# Autodesk Inventor assembly: link1
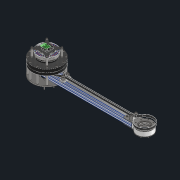
[picture p0: Inventor's stored thumbnail of the model, 180x180]
Saved by Autodesk Inventor 2022 (Build 260153000, 153)
## iProperties
Created: 2021-10-13
Part Number: link1
Document SubType Name: Assembly
Designer: Yuta Kage
Author: Yuta Kage
## Documents named in this file (2)
- C:\Users\yuta0\Documents\GitHub\catchrobo_hardware\mesh\scara\link1.iam
- C:\Users\yuta0\Documents\GitHub\catchrobo_hardware\assy-scara\s-assy-scara_link1.iam
## Components (1 placed, 1 different names)
1. s-assy-scara_link1:1 [sub-assembly] — メイト:1, メイト:2, メイト:3
## Relationships (3: Mate 3)
- メイト:1 [Mate]: s-assy-scara_link1:1
- メイト:2 [Mate]: s-assy-scara_link1:1
- メイト:3 [Mate] (-10 mm): s-assy-scara_link1:1
